# Autodesk Inventor assembly: KB33-046-002 - Привод в сборе зеркальный
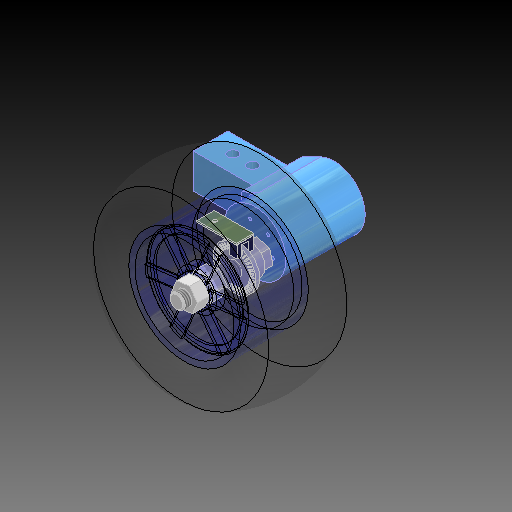
[picture p0: Inventor's stored thumbnail of the model, 512x512]
Saved by Autodesk Inventor 2020 (Build 240168000, 168)
## iProperties
Created: 2021-06-21
Part Number: KB33-046-002 - Привод в сборе зеркальный
Document SubType Name: Assembly
Designer: Петров Иван
Mass: 1177.92 g
Surface Area: 1659.54 cm^2
Volume: 1172.17 cm^3
Density: 1.00491 g/cm^3
Author: Петров Иван
## Documents named in this file (8)
- E:\IVAN\Ivan_desktop\Kvantorium\Projects\RoboPatrol\design\KB33-046-002 - Привод в сборе зеркальный.iam
- E:\IVAN\Ivan_desktop\Kvantorium\Projects\RoboPatrol\design\KB33-046-002-001 - Крепление зеркальный.ipt
- E:\IVAN\Ivan_desktop\Kvantorium\Projects\RoboPatrol\design\standart_components\dc_gear_motor_12V_500rpm\dc_gear_motor_12V_500rpm зеркальный.ipt
- E:\IVAN\Ivan_desktop\Kvantorium\Projects\RoboPatrol\design\standart_components\WheelBig\колесо большое1 зеркальный.iam
- E:\IVAN\Ivan_desktop\Kvantorium\Projects\RoboPatrol\design\KB33-046-002-002 - Втулка зеркальный.ipt
- E:\IVAN\Ivan_desktop\Kvantorium\Projects\RoboPatrol\design\KB33-046-002-003 - Фиксирующая гайка зеркальный.ipt
- E:\IVAN\Ivan_desktop\Kvantorium\Projects\RoboPatrol\design\KB33-046-002-004 - Колесо энкодера зеркальный.ipt
- E:\IVAN\Ivan_desktop\Kvantorium\Projects\RoboPatrol\design\standart_components\Standart optical endstop зеркальный.ipt
## Components (9 placed, 7 different names)
1. KB33-046-002-001 - Крепление зеркальный:1 — Совмещение:2, Совмещение:1, Заподлицо:1, Угол:6
2. dc_gear_motor_12V_500rpm зеркальный:1 — Совмещение:2, Совмещение:1, Заподлицо:1, Совмещение:4, Совмещение:3, Угол:1, Совмещение:6, Совмещение:5
3. колесо большое1 зеркальный:1 [sub-assembly] — Совмещение:4, Совмещение:3, Совмещение:8, Угол:2, Совмещение:10
4. KB33-046-002-002 - Втулка зеркальный:1 — Угол:1, Совмещение:6, Совмещение:5, Совмещение:7, Совмещение:9, Совмещение:12, Угол:3, Совмещение:11, Совмещение:14
5. KB33-046-002-003 - Фиксирующая гайка зеркальный:1 — Совмещение:8, Угол:2, Совмещение:7, Угол:4
6. KB33-046-002-003 - Фиксирующая гайка зеркальный:2 — Угол:4, Совмещение:10, Совмещение:9
7. KB33-046-002-003 - Фиксирующая гайка зеркальный:3 — Совмещение:12, Угол:3, Совмещение:11, Угол:5, Совмещение:13
8. KB33-046-002-004 - Колесо энкодера зеркальный:1 — Угол:5, Совмещение:14, Совмещение:13, Совмещение:15, Касательность:1
9. Standart optical endstop зеркальный:1 — Совмещение:15, Угол:6, Касательность:1
## Relationships (23: Mate 15, Angle 6, Flush 1, Tangent 1)
- Совмещение:2 [Mate]: KB33-046-002-001 - Крепление зеркальный:1 ↔ dc_gear_motor_12V_500rpm зеркальный:1
- Совмещение:1 [Mate]: KB33-046-002-001 - Крепление зеркальный:1 ↔ dc_gear_motor_12V_500rpm зеркальный:1
- Заподлицо:1 [Flush]: KB33-046-002-001 - Крепление зеркальный:1 ↔ dc_gear_motor_12V_500rpm зеркальный:1
- Совмещение:4 [Mate]: dc_gear_motor_12V_500rpm зеркальный:1 ↔ колесо большое1 зеркальный:1
- Совмещение:3 [Mate] (30 mm): dc_gear_motor_12V_500rpm зеркальный:1 ↔ колесо большое1 зеркальный:1
- Угол:1 [Angle] (180 deg): dc_gear_motor_12V_500rpm зеркальный:1 ↔ KB33-046-002-002 - Втулка зеркальный:1
- Совмещение:6 [Mate]: dc_gear_motor_12V_500rpm зеркальный:1 ↔ KB33-046-002-002 - Втулка зеркальный:1
- Совмещение:5 [Mate]: dc_gear_motor_12V_500rpm зеркальный:1 ↔ KB33-046-002-002 - Втулка зеркальный:1
- Совмещение:8 [Mate]: колесо большое1 зеркальный:1 ↔ KB33-046-002-003 - Фиксирующая гайка зеркальный:1
- Угол:2 [Angle] (0 deg): колесо большое1 зеркальный:1 ↔ KB33-046-002-003 - Фиксирующая гайка зеркальный:1
- Совмещение:7 [Mate]: KB33-046-002-002 - Втулка зеркальный:1 ↔ KB33-046-002-003 - Фиксирующая гайка зеркальный:1
- Угол:4 [Angle] (0 deg): KB33-046-002-003 - Фиксирующая гайка зеркальный:1 ↔ KB33-046-002-003 - Фиксирующая гайка зеркальный:2
- Совмещение:10 [Mate]: колесо большое1 зеркальный:1 ↔ KB33-046-002-003 - Фиксирующая гайка зеркальный:2
- Совмещение:9 [Mate]: KB33-046-002-002 - Втулка зеркальный:1 ↔ KB33-046-002-003 - Фиксирующая гайка зеркальный:2
- Совмещение:12 [Mate]: KB33-046-002-002 - Втулка зеркальный:1 ↔ KB33-046-002-003 - Фиксирующая гайка зеркальный:3
- Угол:3 [Angle] (0 deg): KB33-046-002-002 - Втулка зеркальный:1 ↔ KB33-046-002-003 - Фиксирующая гайка зеркальный:3
- Совмещение:11 [Mate]: KB33-046-002-002 - Втулка зеркальный:1 ↔ KB33-046-002-003 - Фиксирующая гайка зеркальный:3
- Угол:5 [Angle] (0 deg): KB33-046-002-003 - Фиксирующая гайка зеркальный:3 ↔ KB33-046-002-004 - Колесо энкодера зеркальный:1
- Совмещение:14 [Mate]: KB33-046-002-002 - Втулка зеркальный:1 ↔ KB33-046-002-004 - Колесо энкодера зеркальный:1
- Совмещение:13 [Mate]: KB33-046-002-003 - Фиксирующая гайка зеркальный:3 ↔ KB33-046-002-004 - Колесо энкодера зеркальный:1
- Совмещение:15 [Mate] (1 mm): KB33-046-002-004 - Колесо энкодера зеркальный:1 ↔ Standart optical endstop зеркальный:1
- Угол:6 [Angle] (270 deg): KB33-046-002-001 - Крепление зеркальный:1 ↔ Standart optical endstop зеркальный:1
- Касательность:1 [Tangent] (3 mm): KB33-046-002-004 - Колесо энкодера зеркальный:1 ↔ Standart optical endstop зеркальный:1
